# Autodesk Inventor assembly: tester
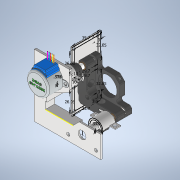
[picture p0: Inventor's stored thumbnail of the model, 180x180]
Saved by Autodesk Inventor 2020.2 (Build 242310000, 310)
## iProperties
Created: 2020-02-18
Part Number: tester
Document SubType Name: Assembly
Designer: ColinP
Author: ColinP
## Documents named in this file (5)
- C:\Users\ColinP\Documents\Inventor\steppermotoriqc\SteppermotorMirror\tester.iam
- C:\Users\ColinP\Documents\Inventor\steppermotoriqc\SteppermotorMirror\Shelf.ipt
- C:\Users\ColinP\Documents\Inventor\steppermotoriqc\SteppermotorMirror\KM100-Step.ipt
- C:\Users\ColinP\Documents\Inventor\steppermotoriqc\SteppermotorMirror\socket.ipt
- C:\Users\ColinP\Documents\Inventor\steppermotoriqc\28BYJ-48 – 5V Stepper Motor\28BYJ-48 – 5V Stepper Motor.ipt
## Components (5 placed, 4 different names)
1. KM100-Step:1 — Mate:1, Mate:2, Angle:1, Mate:3, Insert:1
2. socket:1
3. Shelf:1 — Mate:1, Mate:2, Angle:1, Mate:3, Mate:4, Mate:5, Mate:6
4. 28BYJ-48 – 5V Stepper Motor:1 — Mate:4, Mate:5, Mate:6
5. socket:2 — Insert:1
## Relationships (8: Mate 6, Angle 1, Insert 1)
- Mate:1: KM100-Step:1 ↔ Shelf:1
- Mate:2: KM100-Step:1 ↔ Shelf:1
- Angle:1 (0 deg): KM100-Step:1 ↔ Shelf:1
- Mate:3: KM100-Step:1 ↔ Shelf:1
- Mate:4: Shelf:1 ↔ 28BYJ-48 – 5V Stepper Motor:1
- Mate:5: Shelf:1 ↔ 28BYJ-48 – 5V Stepper Motor:1
- Mate:6: Shelf:1 ↔ 28BYJ-48 – 5V Stepper Motor:1
- Insert:1: KM100-Step:1 ↔ socket:2
